# Autodesk Inventor assembly: SM1_LensBridge
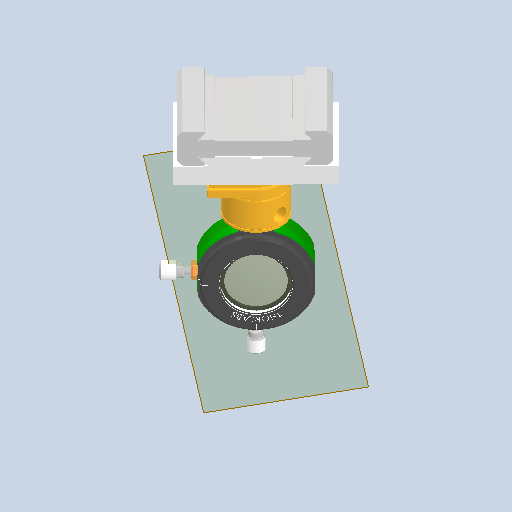
[picture p0: Inventor's stored thumbnail of the model, 512x512]
Saved by Autodesk Inventor 2026.1 (Build 301233000, 233)
## iProperties
Created: 2019-08-20
Part Number: SM1_LensBridge
Document SubType Name: Assembly
Designer: Julian
Author: Julian
## Documents named in this file (7)
- C:\Users\user\Desktop\setup for publishing\SM1_LensBridge_160mm.iam
- C:\Users\user\Desktop\setup for publishing\XT66D2-40-Step_post_mount.ipt
- C:\Users\user\Desktop\setup for publishing\XT66C2-Step_rail mount.ipt
- C:\Users\user\Desktop\setup for publishing\160 mm lens.iam
- C:\Users\user\Desktop\setup for publishing\SM1LensXYmount - grün.ipt
- C:\Users\user\Desktop\setup for publishing\M-PS-KF_miroor_flip.ipt
- C:\Users\user\Desktop\setup for publishing\M-PS-0_5E_0_5in_post+1mm spacer.ipt
## Components (6 placed, 6 different names)
1. XT66D2-40-Step_post_mount:1 — Mate:9, Mate:10, Flush:1, Angle:1, Mate:15, Mate:16, Angle:2
2. XT66C2-Step_rail mount:1 — Mate:9, Mate:10, Flush:1
3. 160 mm lens:1 [sub-assembly] — Mate:13, Mate:14
4. SM1LensXYmount - grün:1 — Angle:1, Mate:13, Mate:14, Mate:19, Mate:20
5. M-PS-KF_miroor_flip:1 — Mate:15, Mate:16, Angle:2, Mate:17, Mate:18
6. M-PS-0_5E_0_5in_post+1mm spacer:1 — Mate:17, Mate:18, Mate:19, Mate:20
## Relationships (13: Mate 10, Angle 2, Flush 1)
- Mate:9: XT66D2-40-Step_post_mount:1 ↔ XT66C2-Step_rail mount:1
- Mate:10: XT66D2-40-Step_post_mount:1 ↔ XT66C2-Step_rail mount:1
- Flush:1: XT66D2-40-Step_post_mount:1 ↔ XT66C2-Step_rail mount:1
- Angle:1 (0 deg): XT66D2-40-Step_post_mount:1 ↔ SM1LensXYmount - grün:1
- Mate:13: 160 mm lens:1 ↔ SM1LensXYmount - grün:1
- Mate:14 (-0.732 mm): 160 mm lens:1 ↔ SM1LensXYmount - grün:1
- Mate:15: XT66D2-40-Step_post_mount:1 ↔ M-PS-KF_miroor_flip:1
- Mate:16: XT66D2-40-Step_post_mount:1 ↔ M-PS-KF_miroor_flip:1
- Angle:2 (0 deg): XT66D2-40-Step_post_mount:1 ↔ M-PS-KF_miroor_flip:1
- Mate:17: M-PS-KF_miroor_flip:1 ↔ M-PS-0_5E_0_5in_post+1mm spacer:1
- Mate:18: M-PS-KF_miroor_flip:1 ↔ M-PS-0_5E_0_5in_post+1mm spacer:1
- Mate:19: SM1LensXYmount - grün:1 ↔ M-PS-0_5E_0_5in_post+1mm spacer:1
- Mate:20: SM1LensXYmount - grün:1 ↔ M-PS-0_5E_0_5in_post+1mm spacer:1
